# Autodesk Inventor assembly: Cerniera Assemb
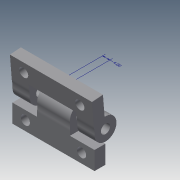
[picture p0: Inventor's stored thumbnail of the model, 180x180]
Saved by Autodesk Inventor 2019 (Build 230136000, 136)
## iProperties
Created: 2019-06-18
Part Number: Cerniera Assemb
Document SubType Name: Assembly
Designer: giacomo
Author: giacomo
## Documents named in this file (3)
- D:\Hobby\Inventor\Prove 3D printer\Cerniera\Cerniera Assemb.iam
- D:\Hobby\Inventor\Prove 3D printer\Cerniera\Cerniera 1.ipt
- D:\Hobby\Inventor\Prove 3D printer\Cerniera\Cerniera 2.ipt
## Components (2 placed, 2 different names)
1. Cerniera 1:1 — Mate:1, Flush:1
2. Cerniera 2:1 — Mate:1, Flush:1
## Relationships (2: Mate 1, Flush 1)
- Mate:1: Cerniera 1:1 ↔ Cerniera 2:1
- Flush:1: Cerniera 1:1 ↔ Cerniera 2:1
